# Autodesk Inventor assembly: Chassis-ver14-1111-2019
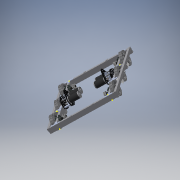
[picture p0: Inventor's stored thumbnail of the model, 180x180]
Saved by Autodesk Inventor 2018 (Build 220112000, 112)
## iProperties
Created: 2019-10-10
Part Number: Chassis-ver14-1111-2019
Document SubType Name: Assembly
Designer: JMHal
Author: JMHal
## Documents named in this file (24)
- E:\GrabCad\2020 Infinite Recharge\Chassis\Assembly\Chassis-ver14-1111-2019.iam
- E:\GrabCad\2020 Infinite Recharge\Chassis\Parts\2x1 20in Alluminum with Cal Drop.ver1-1111-2019.ipt
- E:\GrabCad\2020 Infinite Recharge\Chassis\Parts\2x1 20in Alluminum.ver1-1111-2019.ipt
- E:\GrabCad\2020 Infinite Recharge\Chassis\Parts\2x1 2in Alluminum Block.ver1-1111-2019.ipt
- E:\GrabCad\Resources\VEXpro Resources\Bearings\0.5inHexFlangedBearing(1.125inx0.313in)-1111-2016.ipt
- E:\GrabCad\Resources\VEXpro Resources\Versa Motion\VersaBlockKit-1111-2016.ipt
- E:\GrabCad\Resources\VEXpro Resources\Shafts\0.5inThunderHexShaft(8)-1111-2016.ipt
- E:\GrabCad\Resources\VEXpro Resources\Gearboxes\WCP SS Gearbox\SS-Gearbox.iam
- E:\GrabCad\Resources\VEXpro Resources\Gussets\ChassisGusset-1111-2016.ipt
- E:\GrabCad\2020 Infinite Recharge\Chassis\Parts\ElectricalBoard.ver1-1111-2019.ipt
- E:\GrabCad\Resources\VEXpro Resources\Spacers\0.5inAcetalSpace(0.5inHex)-1111-2016.ipt
- E:\GrabCad\Resources\VEXpro Resources\Spacers\0.5inAcetalSpace(0.5inHex)-1111-2016_MIR.ipt
- E:\GrabCad\Resources\VEXpro Resources\Versa Motion\Timing Pulleys\TimingPulley30T15mmDoubleFlange(0.5inHex)-1111-2017.ipt
- E:\GrabCad\Resources\VEXpro Resources\Spacers\0.25inAcetalSpacer(0.5inHex)-1111-2016.ipt
- E:\GrabCad\Resources\VEXpro Resources\Spacers\1inAcetalSpacer(0.5inHex)-1111-2016.ipt
- E:\GrabCad\Resources\VEXpro Resources\Versa Motion\Timing Pulleys\TimingPulley30T15mmDoubleFlange(0.5inHex)-1111-2017_MIR.ipt
- E:\GrabCad\Resources\VEXpro Resources\Spacers\0.25inAcetalSpacer(0.5inHex)-1111-2016_MIR.ipt
- E:\GrabCad\Resources\VEXpro Resources\Spacers\1inAcetalSpacer(0.5inHex)-1111-2016_MIR.ipt
- E:\GrabCad\Resources\VEXpro Resources\Wheels\6 inch\6x1inTractionWheel-1111-2016.iam
- E:\GrabCad\2020 Infinite Recharge\Chassis\Parts\Bumbers.ver1-1111-2019.ipt
- C:\Users\Demarcus\Desktop\WCDShiftingGearboxPTO.ver1-1111-2020.iam
- E:\GrabCad\Season Archives\2019 - Deep Space\Chassis\Parts\AluminumBracket.ipt
- E:\GrabCad\2020 Infinite Recharge\Chassis\Parts\BumperMount1-ver1-1111-2019.ipt
- E:\GrabCad\2020 Infinite Recharge\Chassis\Parts\AluminumBracket2-ver1-1111-2019.ipt
## Components (73 placed, 23 different names)
1. 2x1 20in Alluminum with Cal Drop.ver1-1111-2019:1 — Mate:31, Mate:32, Insert:8, Mate:53, Angle:9, Insert:19, Angle:11, Flush:1, Mate:65, Mate:66, Flush:2, Mate:77, Mate:78, Flush:16, Flush:17, Mate:80, Flush:20, Flush:23, Symmetry:1, Flush:43, Symmetry:2, Flush:62, Mate:141, Mate:144, Mate:145, Mate:146, Angle:15, Mate:147, Mate:148, Angle:16, Mate:149, Mate:223, Mate:225, Mate:226, Mate:239
2. 2x1 20in Alluminum.ver1-1111-2019:1 — Mate:65, Mate:66, Flush:2, Mate:68, Mate:72, Mate:81, Flush:22, Mate:82, Flush:24, Flush:44, Flush:62, Mate:140, Flush:63, Mate:197, Mate:198, Mate:199, Mate:200, Mate:201, Mate:213, Mate:214, Mate:215, Mate:216
3. 2x1 20in Alluminum with Cal Drop.ver1-1111-2019:2 — Insert:5, Angle:7, Insert:23, Angle:13, Flush:8, Flush:9, Flush:34, Flush:35, Flush:36, Symmetry:1, Symmetry:2, Cylindrical:42, Mate:142, Mate:143, Mate:154, Mate:155, Mate:156, Mate:157, Angle:17, Mate:158, Mate:159, Angle:18, Angle:20, Mate:224, Mate:238, Mate:240
4. 2x1 20in Alluminum.ver1-1111-2019:2 — Mate:223, Mate:224, Mate:225, Mate:226, Mate:227, Mate:228, Mate:229, Mate:230, Mate:231, Mate:233, Mate:234, Mate:236, Mate:237
5. ChassisGusset-1111-2016:1 — Mate:76, Flush:12, Flush:36
6. ChassisGusset-1111-2016:2 — Mate:75, Flush:11, Flush:35
7. ChassisGusset-1111-2016:3 — Mate:78, Flush:14, Flush:17
8. ChassisGusset-1111-2016:4 — Mate:77, Flush:15, Flush:16
9. ChassisGusset-1111-2016:5 — Mate:82, Flush:24, Flush:34
10. ChassisGusset-1111-2016:6 — Mate:81, Flush:22, Flush:23
11. ChassisGusset-1111-2016:7 — Mate:80, Flush:20, Mate:227
12. ElectricalBoard.ver1-1111-2019:1 — Flush:43, Flush:44
13. 0.5inAcetalSpace(0.5inHex)-1111-2016:1 — Cylindrical:59, Mate:202, Cylindrical:60, Mate:203
14. 0.5inAcetalSpace(0.5inHex)-1111-2016_MIR:1 — Cylindrical:53, Mate:193, Cylindrical:54, Mate:194
15. TimingPulley30T15mmDoubleFlange(0.5inHex)-1111-2017:1 — Rotational:7
16. 0.25inAcetalSpacer(0.5inHex)-1111-2016:2 — Rotational:6, Rotational:7
17. 1inAcetalSpacer(0.5inHex)-1111-2016:1 — Rotational:5, Rotational:6
18. TimingPulley30T15mmDoubleFlange(0.5inHex)-1111-2017_MIR:1 — Rotational:10
19. 0.25inAcetalSpacer(0.5inHex)-1111-2016_MIR:2 — Rotational:10, Rotational:11
20. 1inAcetalSpacer(0.5inHex)-1111-2016_MIR:1 — Rotational:11, Rotational:13
21. 6x1inTractionWheel-1111-2016:1 [sub-assembly] — Mate:203, Cylindrical:64, Flush:66
22. 6x1inTractionWheel-1111-2016:5 [sub-assembly] — Cylindrical:55, Mate:194, Flush:65
23. Bumbers.ver1-1111-2019:1 — Mate:139, Mate:140, Mate:208
24. WCDShiftingGearboxPTO.ver1-1111-2020:1 [sub-assembly] — Cylindrical:42
25. SS-Gearbox:3 [sub-assembly] — Mate:144, Mate:145, Cylindrical:51, Mate:204
26. VersaBlockKit-1111-2016:13 — Mate:146, Angle:15, Mate:147, Rotational:17
27. VersaBlockKit-1111-2016:14 — Mate:148, Angle:16, Mate:149, Cylindrical:45, Mate:153
28. 0.5inHexFlangedBearing(1.125inx0.313in)-1111-2016:21 — Cylindrical:45, Mate:153, Cylindrical:61, Mate:205
29. 6x1inTractionWheel-1111-2016:11 [sub-assembly] — Cylindrical:63, Mate:206, Mate:207
30. TimingPulley30T15mmDoubleFlange(0.5inHex)-1111-2017:2 — Cylindrical:46, Rotational:18
31. 0.5inHexFlangedBearing(1.125inx0.313in)-1111-2016:22 — Rotational:17, Cylindrical:47, Mate:166
32. 0.5inAcetalSpace(0.5inHex)-1111-2016_MIR:3 — Cylindrical:46, Mate:150, Mate:151, Rotational:18
33. 1inAcetalSpacer(0.5inHex)-1111-2016_MIR:2 — Mate:150, Mate:151, Cylindrical:47, Mate:166
34. 0.5inAcetalSpace(0.5inHex)-1111-2016:3 — Cylindrical:61, Mate:205, Cylindrical:62, Mate:206
35. SS-Gearbox:4 [sub-assembly] — Mate:154, Mate:155, Cylindrical:52, Angle:20, Mate:192
36. VersaBlockKit-1111-2016:15 — Mate:156, Mate:157, Angle:17, Mate:160, Angle:19
37. VersaBlockKit-1111-2016:16 — Mate:158, Mate:159, Angle:18, Mate:161, Mate:165, Angle:21
38. 0.5inHexFlangedBearing(1.125inx0.313in)-1111-2016:23 — Mate:160, Angle:19, Cylindrical:56, Mate:195
39. 0.5inHexFlangedBearing(1.125inx0.313in)-1111-2016:24 — Mate:161, Rotational:21, Mate:165, Angle:21
40. 1inAcetalSpacer(0.5inHex)-1111-2016_MIR:3 — Mate:162, Mate:163, Rotational:21
41. 0.5inAcetalSpace(0.5inHex)-1111-2016_MIR:4 — Mate:162, Mate:163, Rotational:22
42. TimingPulley30T15mmDoubleFlange(0.5inHex)-1111-2017:3 — Rotational:22
43. 0.5inAcetalSpace(0.5inHex)-1111-2016:4 — Cylindrical:56, Mate:195, Cylindrical:57, Mate:196
44. 0.5inThunderHexShaft(8)-1111-2016:5 — Cylindrical:50, Cylindrical:57, Cylindrical:58
45. 6x1inTractionWheel-1111-2016:12 [sub-assembly] — Cylindrical:50, Cylindrical:58, Mate:196
46. 6x1inTractionWheel-1111-2016:13 [sub-assembly] — Cylindrical:51, Mate:204
47. 6x1inTractionWheel-1111-2016:14 [sub-assembly] — Cylindrical:52, Mate:192
48. AluminumBracket:1 — Mate:167, Mate:168, Mate:169
49. AluminumBracket:4 — Mate:176, Mate:177, Mate:178
50. AluminumBracket:5 — Mate:179, Mate:180, Mate:181
51. AluminumBracket:7 — Mate:185, Mate:186, Mate:187
52. 0.5inThunderHexShaft(8)-1111-2016:6 — Cylindrical:54, Cylindrical:55, Flush:65
53. BumperMount1-ver1-1111-2019:2 — Mate:197, Mate:198, Mate:199, Mate:222, Mate:228, Mate:229, Mate:235
54. BumperMount1-ver1-1111-2019:3 — Mate:200, Mate:201, Mate:208, Mate:221, Mate:232
55. 0.5inThunderHexShaft(8)-1111-2016:7 — Cylindrical:60, Cylindrical:64, Flush:66
56. 0.5inThunderHexShaft(8)-1111-2016:8 — Cylindrical:62, Cylindrical:63, Mate:207
57. AluminumBracket2-ver1-1111-2019:1 — Mate:230, Mate:231, Mate:232
58. AluminumBracket2-ver1-1111-2019:2 — Mate:233, Mate:234, Mate:235
59. AluminumBracket2-ver1-1111-2019:3 — Mate:213, Mate:214, Mate:222
60. AluminumBracket2-ver1-1111-2019:4 — Mate:215, Mate:216, Mate:221
61. ChassisGusset-1111-2016:8 — Mate:236, Mate:237, Mate:238
62. 0.5inHexFlangedBearing(1.125inx0.313in)-1111-2016:19 — Rotational:13
63. 0.5inHexFlangedBearing(1.125inx0.313in)-1111-2016:7 — Insert:5, Mate:48, Mate:49, Cylindrical:53, Mate:193
64. 0.5inHexFlangedBearing(1.125inx0.313in)-1111-2016:17 — Insert:19, Rotational:5
65. 0.5inHexFlangedBearing(1.125inx0.313in)-1111-2016:10 — Insert:8, Mate:52, Cylindrical:59, Mate:202
66. 2x1 2in Alluminum Block.ver1-1111-2019:5 — Mate:31, Mate:32, Flush:15, Mate:167, Mate:168, Mate:169, Mate:239
67. 2x1 2in Alluminum Block.ver1-1111-2019:6 — Flush:1, Mate:68, Flush:14, Mate:141, Mate:176, Mate:177, Mate:178
68. 2x1 2in Alluminum Block.ver1-1111-2019:7 — Mate:72, Flush:9, Mate:75, Flush:11, Mate:143, Flush:63, Mate:179, Mate:180, Mate:181
69. 2x1 2in Alluminum Block.ver1-1111-2019:8 — Flush:8, Mate:76, Flush:12, Mate:139, Mate:142, Mate:185, Mate:186, Mate:187, Mate:240
70. VersaBlockKit-1111-2016:3 — Mate:48, Mate:49, Angle:7
71. VersaBlockKit-1111-2016:6 — Mate:52, Mate:53, Angle:9
72. VersaBlockKit-1111-2016:9 — Angle:11
73. VersaBlockKit-1111-2016:11 — Insert:23, Angle:13
## Relationships (169: Mate 98, Flush 23, CylindricalJoint 19, Angle 11, RevoluteJoint 10, Insert 6, Symmetry 2)
- Mate:31: 2x1 20in Alluminum with Cal Drop.ver1-1111-2019:1 ↔ 2x1 2in Alluminum Block.ver1-1111-2019:5
- Mate:32: 2x1 20in Alluminum with Cal Drop.ver1-1111-2019:1 ↔ 2x1 2in Alluminum Block.ver1-1111-2019:5
- Insert:5: 2x1 20in Alluminum with Cal Drop.ver1-1111-2019:2 ↔ 0.5inHexFlangedBearing(1.125inx0.313in)-1111-2016:7
- Mate:48: 0.5inHexFlangedBearing(1.125inx0.313in)-1111-2016:7 ↔ VersaBlockKit-1111-2016:3
- Mate:49: 0.5inHexFlangedBearing(1.125inx0.313in)-1111-2016:7 ↔ VersaBlockKit-1111-2016:3
- Insert:8: 2x1 20in Alluminum with Cal Drop.ver1-1111-2019:1 ↔ 0.5inHexFlangedBearing(1.125inx0.313in)-1111-2016:10
- Angle:7 (0 deg): 2x1 20in Alluminum with Cal Drop.ver1-1111-2019:2 ↔ VersaBlockKit-1111-2016:3
- Mate:52: 0.5inHexFlangedBearing(1.125inx0.313in)-1111-2016:10 ↔ VersaBlockKit-1111-2016:6
- Mate:53: 2x1 20in Alluminum with Cal Drop.ver1-1111-2019:1 ↔ VersaBlockKit-1111-2016:6
- Angle:9 (0 deg): 2x1 20in Alluminum with Cal Drop.ver1-1111-2019:1 ↔ VersaBlockKit-1111-2016:6
- [Mate]: 0.5inHexFlangedBearing(1.125inx0.313in)-1111-2016:17 ↔ VersaBlockKit-1111-2016:9
- [Insert]: 0.5inHexFlangedBearing(1.125inx0.313in)-1111-2016:17 ↔ VersaBlockKit-1111-2016:9
- Insert:19: 2x1 20in Alluminum with Cal Drop.ver1-1111-2019:1 ↔ 0.5inHexFlangedBearing(1.125inx0.313in)-1111-2016:17
- Angle:11 (0 deg): 2x1 20in Alluminum with Cal Drop.ver1-1111-2019:1 ↔ VersaBlockKit-1111-2016:9
- [Mate]: 0.5inHexFlangedBearing(1.125inx0.313in)-1111-2016:19 ↔ VersaBlockKit-1111-2016:11
- [Insert]: 0.5inHexFlangedBearing(1.125inx0.313in)-1111-2016:19 ↔ VersaBlockKit-1111-2016:11
- Insert:23: 2x1 20in Alluminum with Cal Drop.ver1-1111-2019:2 ↔ VersaBlockKit-1111-2016:11
- Angle:13 (0 deg): 2x1 20in Alluminum with Cal Drop.ver1-1111-2019:2 ↔ VersaBlockKit-1111-2016:11
- Flush:1: 2x1 20in Alluminum with Cal Drop.ver1-1111-2019:1 ↔ 2x1 2in Alluminum Block.ver1-1111-2019:6
- Mate:65: 2x1 20in Alluminum with Cal Drop.ver1-1111-2019:1 ↔ 2x1 20in Alluminum.ver1-1111-2019:1
- Mate:66: 2x1 20in Alluminum with Cal Drop.ver1-1111-2019:1 ↔ 2x1 20in Alluminum.ver1-1111-2019:1
- Flush:2: 2x1 20in Alluminum with Cal Drop.ver1-1111-2019:1 ↔ 2x1 20in Alluminum.ver1-1111-2019:1
- Mate:68 (254 mm): 2x1 20in Alluminum.ver1-1111-2019:1 ↔ 2x1 2in Alluminum Block.ver1-1111-2019:6
- Flush:8: 2x1 20in Alluminum with Cal Drop.ver1-1111-2019:2 ↔ 2x1 2in Alluminum Block.ver1-1111-2019:8
- Mate:72 (254 mm): 2x1 20in Alluminum.ver1-1111-2019:1 ↔ 2x1 2in Alluminum Block.ver1-1111-2019:7
- Flush:9: 2x1 20in Alluminum with Cal Drop.ver1-1111-2019:2 ↔ 2x1 2in Alluminum Block.ver1-1111-2019:7
- Mate:75: ChassisGusset-1111-2016:2 ↔ 2x1 2in Alluminum Block.ver1-1111-2019:7
- Flush:11: ChassisGusset-1111-2016:2 ↔ 2x1 2in Alluminum Block.ver1-1111-2019:7
- Mate:76: ChassisGusset-1111-2016:1 ↔ 2x1 2in Alluminum Block.ver1-1111-2019:8
- Flush:12: ChassisGusset-1111-2016:1 ↔ 2x1 2in Alluminum Block.ver1-1111-2019:8
- Mate:77: 2x1 20in Alluminum with Cal Drop.ver1-1111-2019:1 ↔ ChassisGusset-1111-2016:4
- Mate:78: 2x1 20in Alluminum with Cal Drop.ver1-1111-2019:1 ↔ ChassisGusset-1111-2016:3
- Flush:14: ChassisGusset-1111-2016:3 ↔ 2x1 2in Alluminum Block.ver1-1111-2019:6
- Flush:15: ChassisGusset-1111-2016:4 ↔ 2x1 2in Alluminum Block.ver1-1111-2019:5
- Flush:16: 2x1 20in Alluminum with Cal Drop.ver1-1111-2019:1 ↔ ChassisGusset-1111-2016:4
- Flush:17: 2x1 20in Alluminum with Cal Drop.ver1-1111-2019:1 ↔ ChassisGusset-1111-2016:3
- Mate:80: 2x1 20in Alluminum with Cal Drop.ver1-1111-2019:1 ↔ ChassisGusset-1111-2016:7
- Flush:20: 2x1 20in Alluminum with Cal Drop.ver1-1111-2019:1 ↔ ChassisGusset-1111-2016:7
- Mate:81: 2x1 20in Alluminum.ver1-1111-2019:1 ↔ ChassisGusset-1111-2016:6
- Flush:22: 2x1 20in Alluminum.ver1-1111-2019:1 ↔ ChassisGusset-1111-2016:6
- Flush:23: 2x1 20in Alluminum with Cal Drop.ver1-1111-2019:1 ↔ ChassisGusset-1111-2016:6
- Mate:82: 2x1 20in Alluminum.ver1-1111-2019:1 ↔ ChassisGusset-1111-2016:5
- Flush:24: 2x1 20in Alluminum.ver1-1111-2019:1 ↔ ChassisGusset-1111-2016:5
- Flush:34: 2x1 20in Alluminum with Cal Drop.ver1-1111-2019:2 ↔ ChassisGusset-1111-2016:5
- Flush:35: 2x1 20in Alluminum with Cal Drop.ver1-1111-2019:2 ↔ ChassisGusset-1111-2016:2
- Flush:36: 2x1 20in Alluminum with Cal Drop.ver1-1111-2019:2 ↔ ChassisGusset-1111-2016:1
- Symmetry:1: 2x1 20in Alluminum with Cal Drop.ver1-1111-2019:1 ↔ 2x1 20in Alluminum with Cal Drop.ver1-1111-2019:2
- Flush:43: 2x1 20in Alluminum with Cal Drop.ver1-1111-2019:1 ↔ ElectricalBoard.ver1-1111-2019:1
- Flush:44: 2x1 20in Alluminum.ver1-1111-2019:1 ↔ ElectricalBoard.ver1-1111-2019:1
- Rotational:5 [RevoluteJoint]: 1inAcetalSpacer(0.5inHex)-1111-2016:1 ↔ 0.5inHexFlangedBearing(1.125inx0.313in)-1111-2016:17
- Rotational:6 [RevoluteJoint]: 0.25inAcetalSpacer(0.5inHex)-1111-2016:2 ↔ 1inAcetalSpacer(0.5inHex)-1111-2016:1
- Rotational:7 [RevoluteJoint]: TimingPulley30T15mmDoubleFlange(0.5inHex)-1111-2017:1 ↔ 0.25inAcetalSpacer(0.5inHex)-1111-2016:2
- Symmetry:2: 2x1 20in Alluminum with Cal Drop.ver1-1111-2019:1 ↔ 2x1 20in Alluminum with Cal Drop.ver1-1111-2019:2
- Rotational:10 [RevoluteJoint]: TimingPulley30T15mmDoubleFlange(0.5inHex)-1111-2017_MIR:1 ↔ 0.25inAcetalSpacer(0.5inHex)-1111-2016_MIR:2
- Rotational:11 [RevoluteJoint]: 0.25inAcetalSpacer(0.5inHex)-1111-2016_MIR:2 ↔ 1inAcetalSpacer(0.5inHex)-1111-2016_MIR:1
- Rotational:13 [RevoluteJoint]: 1inAcetalSpacer(0.5inHex)-1111-2016_MIR:1 ↔ 0.5inHexFlangedBearing(1.125inx0.313in)-1111-2016:19
- Flush:62 (69.85 mm): 2x1 20in Alluminum with Cal Drop.ver1-1111-2019:1 ↔ 2x1 20in Alluminum.ver1-1111-2019:1
- Mate:139 (-127 mm): Bumbers.ver1-1111-2019:1 ↔ 2x1 2in Alluminum Block.ver1-1111-2019:8
- Mate:140: 2x1 20in Alluminum.ver1-1111-2019:1 ↔ Bumbers.ver1-1111-2019:1
- Cylindrical:42: 2x1 20in Alluminum with Cal Drop.ver1-1111-2019:2 ↔ WCDShiftingGearboxPTO.ver1-1111-2020:1
- Mate:141: 2x1 20in Alluminum with Cal Drop.ver1-1111-2019:1 ↔ 2x1 2in Alluminum Block.ver1-1111-2019:6
- Mate:142: 2x1 20in Alluminum with Cal Drop.ver1-1111-2019:2 ↔ 2x1 2in Alluminum Block.ver1-1111-2019:8
- Mate:143: 2x1 20in Alluminum with Cal Drop.ver1-1111-2019:2 ↔ 2x1 2in Alluminum Block.ver1-1111-2019:7
- Flush:63: 2x1 20in Alluminum.ver1-1111-2019:1 ↔ 2x1 2in Alluminum Block.ver1-1111-2019:7
- Mate:144: 2x1 20in Alluminum with Cal Drop.ver1-1111-2019:1 ↔ SS-Gearbox:3
- Mate:145: 2x1 20in Alluminum with Cal Drop.ver1-1111-2019:1 ↔ SS-Gearbox:3
- Mate:146: 2x1 20in Alluminum with Cal Drop.ver1-1111-2019:1 ↔ VersaBlockKit-1111-2016:13
- Angle:15 (0 deg): 2x1 20in Alluminum with Cal Drop.ver1-1111-2019:1 ↔ VersaBlockKit-1111-2016:13
- Mate:147: 2x1 20in Alluminum with Cal Drop.ver1-1111-2019:1 ↔ VersaBlockKit-1111-2016:13
- Mate:148: 2x1 20in Alluminum with Cal Drop.ver1-1111-2019:1 ↔ VersaBlockKit-1111-2016:14
- Angle:16 (0 deg): 2x1 20in Alluminum with Cal Drop.ver1-1111-2019:1 ↔ VersaBlockKit-1111-2016:14
- Mate:149: 2x1 20in Alluminum with Cal Drop.ver1-1111-2019:1 ↔ VersaBlockKit-1111-2016:14
- Cylindrical:45: VersaBlockKit-1111-2016:14 ↔ 0.5inHexFlangedBearing(1.125inx0.313in)-1111-2016:21
- Rotational:17 [RevoluteJoint]: VersaBlockKit-1111-2016:13 ↔ 0.5inHexFlangedBearing(1.125inx0.313in)-1111-2016:22
- Cylindrical:46: TimingPulley30T15mmDoubleFlange(0.5inHex)-1111-2017:2 ↔ 0.5inAcetalSpace(0.5inHex)-1111-2016_MIR:3
- Mate:150: 0.5inAcetalSpace(0.5inHex)-1111-2016_MIR:3 ↔ 1inAcetalSpacer(0.5inHex)-1111-2016_MIR:2
- Mate:151: 0.5inAcetalSpace(0.5inHex)-1111-2016_MIR:3 ↔ 1inAcetalSpacer(0.5inHex)-1111-2016_MIR:2
- Cylindrical:47: 0.5inHexFlangedBearing(1.125inx0.313in)-1111-2016:22 ↔ 1inAcetalSpacer(0.5inHex)-1111-2016_MIR:2
- Rotational:18 [RevoluteJoint] (7.9375 mm): TimingPulley30T15mmDoubleFlange(0.5inHex)-1111-2017:2 ↔ 0.5inAcetalSpace(0.5inHex)-1111-2016_MIR:3
- Mate:153: VersaBlockKit-1111-2016:14 ↔ 0.5inHexFlangedBearing(1.125inx0.313in)-1111-2016:21
- Mate:154: 2x1 20in Alluminum with Cal Drop.ver1-1111-2019:2 ↔ SS-Gearbox:4
- Mate:155: 2x1 20in Alluminum with Cal Drop.ver1-1111-2019:2 ↔ SS-Gearbox:4
- Mate:156: 2x1 20in Alluminum with Cal Drop.ver1-1111-2019:2 ↔ VersaBlockKit-1111-2016:15
- Mate:157: 2x1 20in Alluminum with Cal Drop.ver1-1111-2019:2 ↔ VersaBlockKit-1111-2016:15
- Angle:17 (0 deg): 2x1 20in Alluminum with Cal Drop.ver1-1111-2019:2 ↔ VersaBlockKit-1111-2016:15
- Mate:158: 2x1 20in Alluminum with Cal Drop.ver1-1111-2019:2 ↔ VersaBlockKit-1111-2016:16
- Mate:159: 2x1 20in Alluminum with Cal Drop.ver1-1111-2019:2 ↔ VersaBlockKit-1111-2016:16
- Angle:18 (0 deg): 2x1 20in Alluminum with Cal Drop.ver1-1111-2019:2 ↔ VersaBlockKit-1111-2016:16
- Mate:160: VersaBlockKit-1111-2016:15 ↔ 0.5inHexFlangedBearing(1.125inx0.313in)-1111-2016:23
- Mate:161: VersaBlockKit-1111-2016:16 ↔ 0.5inHexFlangedBearing(1.125inx0.313in)-1111-2016:24
- Angle:19 (0 deg): VersaBlockKit-1111-2016:15 ↔ 0.5inHexFlangedBearing(1.125inx0.313in)-1111-2016:23
- Mate:162: 1inAcetalSpacer(0.5inHex)-1111-2016_MIR:3 ↔ 0.5inAcetalSpace(0.5inHex)-1111-2016_MIR:4
- Mate:163: 1inAcetalSpacer(0.5inHex)-1111-2016_MIR:3 ↔ 0.5inAcetalSpace(0.5inHex)-1111-2016_MIR:4
- Rotational:21 [RevoluteJoint]: 0.5inHexFlangedBearing(1.125inx0.313in)-1111-2016:24 ↔ 1inAcetalSpacer(0.5inHex)-1111-2016_MIR:3
- Rotational:22 [RevoluteJoint] (-7.9375 mm): 0.5inAcetalSpace(0.5inHex)-1111-2016_MIR:4 ↔ TimingPulley30T15mmDoubleFlange(0.5inHex)-1111-2017:3
- Cylindrical:50: 0.5inThunderHexShaft(8)-1111-2016:5 ↔ 6x1inTractionWheel-1111-2016:12
- Cylindrical:51: SS-Gearbox:3 ↔ 6x1inTractionWheel-1111-2016:13
- Cylindrical:52: SS-Gearbox:4 ↔ 6x1inTractionWheel-1111-2016:14
- Angle:20 (90 deg): 2x1 20in Alluminum with Cal Drop.ver1-1111-2019:2 ↔ SS-Gearbox:4
- Mate:165: VersaBlockKit-1111-2016:16 ↔ 0.5inHexFlangedBearing(1.125inx0.313in)-1111-2016:24
- Angle:21 (0 deg): VersaBlockKit-1111-2016:16 ↔ 0.5inHexFlangedBearing(1.125inx0.313in)-1111-2016:24
- Mate:166: 0.5inHexFlangedBearing(1.125inx0.313in)-1111-2016:22 ↔ 1inAcetalSpacer(0.5inHex)-1111-2016_MIR:2
- Mate:167: AluminumBracket:1 ↔ 2x1 2in Alluminum Block.ver1-1111-2019:5
- Mate:168: AluminumBracket:1 ↔ 2x1 2in Alluminum Block.ver1-1111-2019:5
- Mate:169: AluminumBracket:1 ↔ 2x1 2in Alluminum Block.ver1-1111-2019:5
- Mate:176: AluminumBracket:4 ↔ 2x1 2in Alluminum Block.ver1-1111-2019:6
- Mate:177: AluminumBracket:4 ↔ 2x1 2in Alluminum Block.ver1-1111-2019:6
- Mate:178 (0.127 mm): AluminumBracket:4 ↔ 2x1 2in Alluminum Block.ver1-1111-2019:6
- Mate:179: AluminumBracket:5 ↔ 2x1 2in Alluminum Block.ver1-1111-2019:7
- Mate:180: AluminumBracket:5 ↔ 2x1 2in Alluminum Block.ver1-1111-2019:7
- Mate:181 (0.0762 mm): AluminumBracket:5 ↔ 2x1 2in Alluminum Block.ver1-1111-2019:7
- Mate:185: AluminumBracket:7 ↔ 2x1 2in Alluminum Block.ver1-1111-2019:8
- Mate:186: AluminumBracket:7 ↔ 2x1 2in Alluminum Block.ver1-1111-2019:8
- Mate:187 (0.6096 mm): AluminumBracket:7 ↔ 2x1 2in Alluminum Block.ver1-1111-2019:8
- Mate:192 (6.35 mm): SS-Gearbox:4 ↔ 6x1inTractionWheel-1111-2016:14
- Cylindrical:53: 0.5inAcetalSpace(0.5inHex)-1111-2016_MIR:1 ↔ 0.5inHexFlangedBearing(1.125inx0.313in)-1111-2016:7
- Mate:193 (6.35 mm): 0.5inAcetalSpace(0.5inHex)-1111-2016_MIR:1 ↔ 0.5inHexFlangedBearing(1.125inx0.313in)-1111-2016:7
- Cylindrical:54: 0.5inAcetalSpace(0.5inHex)-1111-2016_MIR:1 ↔ 0.5inThunderHexShaft(8)-1111-2016:6
- Cylindrical:55: 6x1inTractionWheel-1111-2016:5 ↔ 0.5inThunderHexShaft(8)-1111-2016:6
- Mate:194: 0.5inAcetalSpace(0.5inHex)-1111-2016_MIR:1 ↔ 6x1inTractionWheel-1111-2016:5
- Cylindrical:56: 0.5inHexFlangedBearing(1.125inx0.313in)-1111-2016:23 ↔ 0.5inAcetalSpace(0.5inHex)-1111-2016:4
- Mate:195 (6.35 mm): 0.5inHexFlangedBearing(1.125inx0.313in)-1111-2016:23 ↔ 0.5inAcetalSpace(0.5inHex)-1111-2016:4
- Cylindrical:57: 0.5inAcetalSpace(0.5inHex)-1111-2016:4 ↔ 0.5inThunderHexShaft(8)-1111-2016:5
- Flush:65 (0.2794 mm): 6x1inTractionWheel-1111-2016:5 ↔ 0.5inThunderHexShaft(8)-1111-2016:6
- Cylindrical:58: 0.5inThunderHexShaft(8)-1111-2016:5 ↔ 6x1inTractionWheel-1111-2016:12
- Mate:196: 0.5inAcetalSpace(0.5inHex)-1111-2016:4 ↔ 6x1inTractionWheel-1111-2016:12
- Mate:197: 2x1 20in Alluminum.ver1-1111-2019:1 ↔ BumperMount1-ver1-1111-2019:2
- Mate:198: 2x1 20in Alluminum.ver1-1111-2019:1 ↔ BumperMount1-ver1-1111-2019:2
- Mate:199: 2x1 20in Alluminum.ver1-1111-2019:1 ↔ BumperMount1-ver1-1111-2019:2
- Mate:200: 2x1 20in Alluminum.ver1-1111-2019:1 ↔ BumperMount1-ver1-1111-2019:3
- Mate:201: 2x1 20in Alluminum.ver1-1111-2019:1 ↔ BumperMount1-ver1-1111-2019:3
- Cylindrical:59: 0.5inAcetalSpace(0.5inHex)-1111-2016:1 ↔ 0.5inHexFlangedBearing(1.125inx0.313in)-1111-2016:10
- Mate:202 (6.35 mm): 0.5inAcetalSpace(0.5inHex)-1111-2016:1 ↔ 0.5inHexFlangedBearing(1.125inx0.313in)-1111-2016:10
- Cylindrical:60: 0.5inAcetalSpace(0.5inHex)-1111-2016:1 ↔ 0.5inThunderHexShaft(8)-1111-2016:7
- Mate:203: 0.5inAcetalSpace(0.5inHex)-1111-2016:1 ↔ 6x1inTractionWheel-1111-2016:1
- Mate:204 (6.35 mm): SS-Gearbox:3 ↔ 6x1inTractionWheel-1111-2016:13
- Cylindrical:61: 0.5inHexFlangedBearing(1.125inx0.313in)-1111-2016:21 ↔ 0.5inAcetalSpace(0.5inHex)-1111-2016:3
- Mate:205 (6.35 mm): 0.5inHexFlangedBearing(1.125inx0.313in)-1111-2016:21 ↔ 0.5inAcetalSpace(0.5inHex)-1111-2016:3
- Cylindrical:62: 0.5inAcetalSpace(0.5inHex)-1111-2016:3 ↔ 0.5inThunderHexShaft(8)-1111-2016:8
- Cylindrical:63: 6x1inTractionWheel-1111-2016:11 ↔ 0.5inThunderHexShaft(8)-1111-2016:8
- Mate:206: 6x1inTractionWheel-1111-2016:11 ↔ 0.5inAcetalSpace(0.5inHex)-1111-2016:3
- Mate:207: 6x1inTractionWheel-1111-2016:11 ↔ 0.5inThunderHexShaft(8)-1111-2016:8
- Mate:208: Bumbers.ver1-1111-2019:1 ↔ BumperMount1-ver1-1111-2019:3
- Mate:213: 2x1 20in Alluminum.ver1-1111-2019:1 ↔ AluminumBracket2-ver1-1111-2019:3
- Mate:214: 2x1 20in Alluminum.ver1-1111-2019:1 ↔ AluminumBracket2-ver1-1111-2019:3
- Mate:215: 2x1 20in Alluminum.ver1-1111-2019:1 ↔ AluminumBracket2-ver1-1111-2019:4
- Mate:216: 2x1 20in Alluminum.ver1-1111-2019:1 ↔ AluminumBracket2-ver1-1111-2019:4
- Mate:221 (230.3145 mm): BumperMount1-ver1-1111-2019:3 ↔ AluminumBracket2-ver1-1111-2019:4
- Mate:222 (230.3145 mm): BumperMount1-ver1-1111-2019:2 ↔ AluminumBracket2-ver1-1111-2019:3
- Mate:223: 2x1 20in Alluminum with Cal Drop.ver1-1111-2019:1 ↔ 2x1 20in Alluminum.ver1-1111-2019:2
- Mate:224: 2x1 20in Alluminum with Cal Drop.ver1-1111-2019:2 ↔ 2x1 20in Alluminum.ver1-1111-2019:2
- Mate:225: 2x1 20in Alluminum with Cal Drop.ver1-1111-2019:1 ↔ 2x1 20in Alluminum.ver1-1111-2019:2
- Mate:226 (69.85 mm): 2x1 20in Alluminum with Cal Drop.ver1-1111-2019:1 ↔ 2x1 20in Alluminum.ver1-1111-2019:2
- Mate:227: 2x1 20in Alluminum.ver1-1111-2019:2 ↔ ChassisGusset-1111-2016:7
- Mate:228: 2x1 20in Alluminum.ver1-1111-2019:2 ↔ BumperMount1-ver1-1111-2019:2
- Mate:229: 2x1 20in Alluminum.ver1-1111-2019:2 ↔ BumperMount1-ver1-1111-2019:2
- Mate:230: 2x1 20in Alluminum.ver1-1111-2019:2 ↔ AluminumBracket2-ver1-1111-2019:1
- Mate:231: 2x1 20in Alluminum.ver1-1111-2019:2 ↔ AluminumBracket2-ver1-1111-2019:1
- Mate:232 (230.3145 mm): BumperMount1-ver1-1111-2019:3 ↔ AluminumBracket2-ver1-1111-2019:1
- Mate:233: 2x1 20in Alluminum.ver1-1111-2019:2 ↔ AluminumBracket2-ver1-1111-2019:2
- Mate:234: 2x1 20in Alluminum.ver1-1111-2019:2 ↔ AluminumBracket2-ver1-1111-2019:2
- Mate:235 (230.3145 mm): BumperMount1-ver1-1111-2019:2 ↔ AluminumBracket2-ver1-1111-2019:2
- Mate:236: 2x1 20in Alluminum.ver1-1111-2019:2 ↔ ChassisGusset-1111-2016:8
- Mate:237: 2x1 20in Alluminum.ver1-1111-2019:2 ↔ ChassisGusset-1111-2016:8
- Mate:238: 2x1 20in Alluminum with Cal Drop.ver1-1111-2019:2 ↔ ChassisGusset-1111-2016:8
- Cylindrical:64: 6x1inTractionWheel-1111-2016:1 ↔ 0.5inThunderHexShaft(8)-1111-2016:7
- Flush:66 (0.1016 mm): 6x1inTractionWheel-1111-2016:1 ↔ 0.5inThunderHexShaft(8)-1111-2016:7
- Mate:239 (279.4 mm): 2x1 20in Alluminum with Cal Drop.ver1-1111-2019:1 ↔ 2x1 2in Alluminum Block.ver1-1111-2019:5
- Mate:240 (254 mm): 2x1 20in Alluminum with Cal Drop.ver1-1111-2019:2 ↔ 2x1 2in Alluminum Block.ver1-1111-2019:8
## Named parameters: d93_d89_d76 = 0 mm, d94_d90 = 0 mm, d103_d89_d76 = 0 mm, d104_d90 = 0 mm
